# Autodesk Inventor assembly: tail_p2
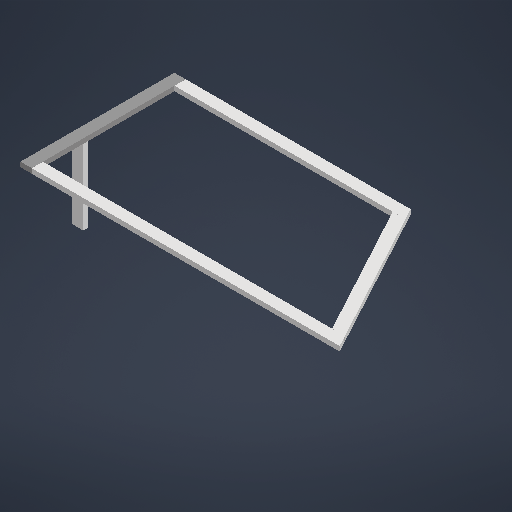
[picture p0: Inventor's stored thumbnail of the model, 512x512]
Saved by Autodesk Inventor 2027.1 (Build 311270010, 270A)
## iProperties
Created: 2026-09-01
Part Number: tail_p2
Document SubType Name: Assembly
Designer: jorda
Author: jorda
## Documents named in this file (6)
- C:\Users\jorda\OneDrive\Documents\GitHub\USC-ASME-TigerBurn-2026\CAD\Tail\tail_p2.iam
- C:\Users\jorda\OneDrive\Documents\GitHub\USC-ASME-TigerBurn-2026\CAD\Tail\2x4x48.ipt
- C:\Users\jorda\OneDrive\Documents\GitHub\USC-ASME-TigerBurn-2026\CAD\Tail\S_2x4x50.56.ipt
- C:\Users\jorda\OneDrive\Documents\GitHub\USC-ASME-TigerBurn-2026\CAD\Tail\S_2x4x72.ipt
- C:\Users\jorda\OneDrive\Documents\GitHub\USC-ASME-TigerBurn-2026\CAD\Tail\S_2x4x96.ipt
- C:\Users\jorda\OneDrive\Documents\GitHub\USC-ASME-TigerBurn-2026\CAD\Tail\2x4x24.ipt
## Components (5 placed, 5 different names)
1. 2x4x48:1 — Mate:3
2. S_2x4x50.56:1
3. S_2x4x72:1
4. S_2x4x96:1
5. 2x4x24:1 — Mate:3
## Relationships (7: Flush 4, Mate 3)
- [Mate]: 2x4x48:1 ↔ S_2x4x72:1
- [Flush]: 2x4x48:1 ↔ S_2x4x72:1
- [Flush]: 2x4x48:1 ↔ S_2x4x72:1
- [Mate]: 2x4x48:1 ↔ S_2x4x96:1
- [Flush]: 2x4x48:1 ↔ S_2x4x96:1
- [Flush]: 2x4x48:1 ↔ S_2x4x96:1
- Mate:3: 2x4x48:1 ↔ 2x4x24:1
